# Autodesk Inventor assembly: rightarm
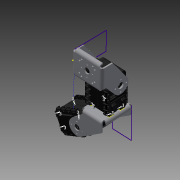
[picture p0: Inventor's stored thumbnail of the model, 180x180]
Saved by Autodesk Inventor 2013 (Build 170138000, 138)
## iProperties
Created: 2014-11-26
Part Number: rightarm
Document SubType Name: Assembly
Designer: Master
Author: Master
## Documents named in this file (3)
- C:\Users\73515\Downloads\DIY-HR-OS1-masterperson40\DIY-HR-OS1-masterperson40\CAD Files\rightarm.iam
- C:\Users\73515\Downloads\DIY-HR-OS1-masterperson40\DIY-HR-OS1-masterperson40\CAD Files\45angle.ipt
- C:\Users\73515\Downloads\DIY-HR-OS1-masterperson40\DIY-HR-OS1-masterperson40\CAD Files\AX12\AX12.iam
## Components (4 placed, 2 different names)
1. 45angle:1 — Mate:1, Mate:2
2. AX12:1 [sub-assembly] — Mate:1, Mate:2, Mate:9, Mate:10, Mate:11
3. 45angle:2 — Mate:7, Mate:8, Mate:9, Mate:10, Mate:11
4. AX12:2 [sub-assembly] — Mate:7, Mate:8
## Relationships (7: Mate 7)
- Mate:1: 45angle:1 ↔ AX12:1
- Mate:2: 45angle:1 ↔ AX12:1
- Mate:7: 45angle:2 ↔ AX12:2
- Mate:8: 45angle:2 ↔ AX12:2
- Mate:9: AX12:1 ↔ 45angle:2
- Mate:10: AX12:1 ↔ 45angle:2
- Mate:11: AX12:1 ↔ 45angle:2
